# Autodesk Inventor assembly: cum_holder_asembly
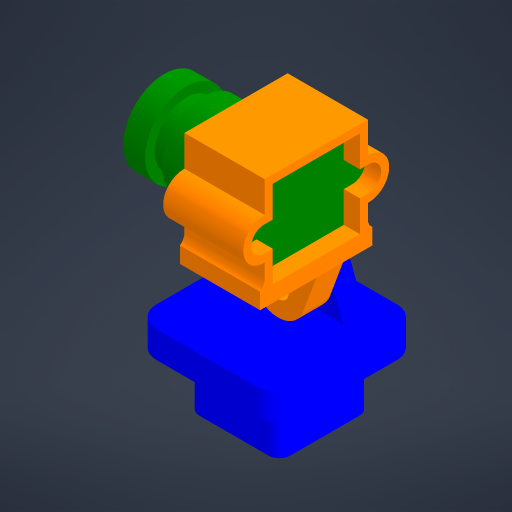
[picture p0: Inventor's stored thumbnail of the model, 512x512]
Saved by Autodesk Inventor 2024 (Build 280153000, 153)
## iProperties
Created: 2023-05-16
Part Number: cum_holder_asembly
Document SubType Name: Assembly
Designer: user
Author: user
## Documents named in this file (4)
- D:\Docs\Robot\3d\machine_body\cum_holder_asembly.iam
- D:\Docs\Robot\3d\machine_body\cum_holder\cum_holder_down.ipt
- D:\Docs\Robot\3d\machine_body\cum_holder\cum_holder_up.ipt
- D:\Docs\Robot\3d\electronics\cum.ipt
## Components (3 placed, 3 different names)
1. cum_holder_down:1 — Заподлицо:1, Заподлицо:2, Совмещение:1, Совмещение:2, Заподлицо:3
2. cum_holder_up:1 — Заподлицо:3, Совмещение:3, Жесткий:1
3. cum:1 — Совмещение:3, Жесткий:1
## Relationships (7: Flush 3, Mate 3, WeldJoint 1)
- Заподлицо:1 [Flush]: cum_holder_down:1
- Заподлицо:2 [Flush]: cum_holder_down:1
- Совмещение:1 [Mate]: cum_holder_down:1
- Совмещение:2 [Mate]: cum_holder_down:1
- Заподлицо:3 [Flush]: cum_holder_down:1 ↔ cum_holder_up:1
- Совмещение:3 [Mate]: cum_holder_up:1 ↔ cum:1
- Жесткий:1 [WeldJoint] (-3 mm): cum_holder_up:1 ↔ cum:1
